# Autodesk Inventor assembly: claws_endeffector_6
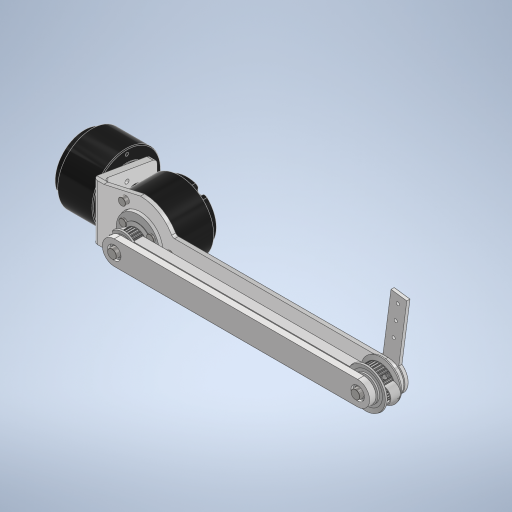
[picture p0: Inventor's stored thumbnail of the model, 512x512]
Saved by Autodesk Inventor 2024 (Build 280153000, 153)
## iProperties
Created: 2025-04-20
Part Number: claws_endeffector_6
Document SubType Name: Assembly
Designer: 1412z
Author: 1412z
## Documents named in this file (17)
- C:\Users\1412z\OneDrive\デスクトップ\rdclab\harvesting_robot\harvesting_endeffector\claws_endeffector\claws_endeffector_6.iam
- C:\Users\1412z\OneDrive\デスクトップ\rdclab\harvesting_robot\harvesting_endeffector\claws_endeffector\motor_holder\motor_holder_6.ipt
- C:\Users\1412z\OneDrive\デスクトップ\rdclab\harvesting_robot\harvesting_endeffector\claws_endeffector\GIM3505-08\GIM3505-8_with-driver.ipt
- C:\Users\1412z\OneDrive\デスクトップ\rdclab\harvesting_robot\harvesting_endeffector\claws_endeffector\misumi\SFL674ZZ_Autodesk_Inventor_2024_20250304\SFL674ZZ.ipt
- C:\Users\1412z\OneDrive\デスクトップ\rdclab\harvesting_robot\harvesting_endeffector\claws_endeffector\misumi\simring\simring_Φ4-Φ5.ipt
- C:\Users\1412z\OneDrive\デスクトップ\rdclab\harvesting_robot\harvesting_endeffector\claws_endeffector\misumi\HTPA22S2M060-A-H4_Autodesk_Inventor_2024_20250419\AIS2024\HTPA22S2M060-A-H4_a-2.ipt
- C:\Users\1412z\OneDrive\デスクトップ\rdclab\harvesting_robot\harvesting_endeffector\claws_endeffector\misumi\M2.5×4\M2.5×4.ipt
- C:\Users\1412z\OneDrive\デスクトップ\rdclab\harvesting_robot\harvesting_endeffector\claws_endeffector\misumi\washer\washer_M4.ipt
- C:\Users\1412z\OneDrive\デスクトップ\rdclab\harvesting_robot\harvesting_endeffector\claws_endeffector\misumi\HTPA32S2M060-A-P4_Autodesk_Inventor_2024_20250419\AIS2024\HTPA32S2M060-A-P4.iam
- C:\Users\1412z\OneDrive\デスクトップ\rdclab\harvesting_robot\harvesting_endeffector\claws_endeffector\motor_holder\motor_holder_top_2.ipt
- C:\Users\1412z\OneDrive\デスクトップ\rdclab\harvesting_robot\harvesting_endeffector\claws_endeffector\cutter_part\cutter_board-2.ipt
- C:\Users\1412z\OneDrive\デスクトップ\rdclab\harvesting_robot\harvesting_endeffector\claws_endeffector\cutter_part\homemade_setcolor-2.ipt
- C:\Users\1412z\OneDrive\デスクトップ\rdclab\harvesting_robot\harvesting_endeffector\claws_endeffector\misumi\shaft\shaft_11.35mm.ipt
- C:\Users\1412z\OneDrive\デスクトップ\rdclab\harvesting_robot\harvesting_endeffector\claws_endeffector\misumi\shaft\shaft_23.3mm.ipt
- C:\Users\1412z\OneDrive\デスクトップ\rdclab\harvesting_robot\harvesting_endeffector\claws_endeffector\misumi\M3×8\M3×8.ipt
- C:\Users\1412z\OneDrive\デスクトップ\rdclab\harvesting_robot\harvesting_endeffector\claws_endeffector\misumi\M3×4\M3×4.ipt
- C:\Users\1412z\OneDrive\デスクトップ\rdclab\harvesting_robot\harvesting_endeffector\claws_endeffector\misumi\HTBN360S2M-60_Inventor\HTBN360S2M-60.ipt
## Components (27 placed, 16 different names)
1. motor_holder_6:1 — 回転:1, 回転:2, 回転:3, 回転:4, 回転:5, 回転:9, 回転:10, 回転:11, 回転:15
2. GIM3505-8_with-driver:1 — 回転:1, 回転:2, 回転:7, 回転:8
3. GIM3505-8_with-driver:2 — 回転:3, 回転:4
4. SFL674ZZ:1 — 回転:5, 回転:6
5. simring_Φ4-Φ5:1 — 回転:6, 回転:23
6. HTPA22S2M060-A-H4_a-2:1 — 回転:7, 回転:8, 回転:12, 回転:13, 回転:14, 回転:18, 回転:30
7. M2.5×4:1 — 回転:10
8. M2.5×4:2 — 回転:12
9. M2.5×4:3 — 回転:14
10. M2.5×4:4 — 回転:11
11. M2.5×4:5 — 回転:13
12. M2.5×4:6 — 回転:9
13. washer_M4:1 — 回転:15, 回転:16
14. HTPA32S2M060-A-P4:1 [sub-assembly] — 回転:16, 回転:17
15. washer_M4:2 — 回転:17, 回転:19
16. washer_M4:3 — 回転:18, 回転:20
17. motor_holder_top_2:1 — 回転:19, 回転:20, 回転:21, 回転:22
18. SFL674ZZ:3 — 回転:21
19. SFL674ZZ:4 — 回転:22, 回転:27
20. cutter_board-2:1 — 回転:23, 回転:24, 回転:25
21. homemade_setcolor-2:1 — 回転:24, 回転:25, 回転:26
22. shaft_11.35mm:1 — 回転:27, 回転:29
23. shaft_23.3mm:1 — 回転:26, 回転:28
24. M3×8:1 — 回転:28
25. M3×4:1 — 回転:29
26. M3×4:2 — 回転:30
27. HTBN360S2M-60:1
## Relationships (30: RevoluteJoint 30)
- 回転:1 [RevoluteJoint]: motor_holder_6:1 ↔ GIM3505-8_with-driver:1
- 回転:2 [RevoluteJoint]: motor_holder_6:1 ↔ GIM3505-8_with-driver:1
- 回転:3 [RevoluteJoint]: motor_holder_6:1 ↔ GIM3505-8_with-driver:2
- 回転:4 [RevoluteJoint]: motor_holder_6:1 ↔ GIM3505-8_with-driver:2
- 回転:5 [RevoluteJoint]: motor_holder_6:1 ↔ SFL674ZZ:1
- 回転:6 [RevoluteJoint]: SFL674ZZ:1 ↔ simring_Φ4-Φ5:1
- 回転:7 [RevoluteJoint]: GIM3505-8_with-driver:1 ↔ HTPA22S2M060-A-H4_a-2:1
- 回転:8 [RevoluteJoint]: GIM3505-8_with-driver:1 ↔ HTPA22S2M060-A-H4_a-2:1
- 回転:9 [RevoluteJoint]: motor_holder_6:1 ↔ M2.5×4:6
- 回転:10 [RevoluteJoint]: motor_holder_6:1 ↔ M2.5×4:1
- 回転:11 [RevoluteJoint]: motor_holder_6:1 ↔ M2.5×4:4
- 回転:12 [RevoluteJoint]: HTPA22S2M060-A-H4_a-2:1 ↔ M2.5×4:2
- 回転:13 [RevoluteJoint]: HTPA22S2M060-A-H4_a-2:1 ↔ M2.5×4:5
- 回転:14 [RevoluteJoint]: HTPA22S2M060-A-H4_a-2:1 ↔ M2.5×4:3
- 回転:15 [RevoluteJoint]: motor_holder_6:1 ↔ washer_M4:1
- 回転:16 [RevoluteJoint]: washer_M4:1 ↔ HTPA32S2M060-A-P4:1
- 回転:17 [RevoluteJoint]: HTPA32S2M060-A-P4:1 ↔ washer_M4:2
- 回転:18 [RevoluteJoint]: HTPA22S2M060-A-H4_a-2:1 ↔ washer_M4:3
- 回転:19 [RevoluteJoint]: washer_M4:2 ↔ motor_holder_top_2:1
- 回転:20 [RevoluteJoint]: washer_M4:3 ↔ motor_holder_top_2:1
- 回転:21 [RevoluteJoint]: motor_holder_top_2:1 ↔ SFL674ZZ:3
- 回転:22 [RevoluteJoint]: motor_holder_top_2:1 ↔ SFL674ZZ:4
- 回転:23 [RevoluteJoint]: simring_Φ4-Φ5:1 ↔ cutter_board-2:1
- 回転:24 [RevoluteJoint]: cutter_board-2:1 ↔ homemade_setcolor-2:1
- 回転:25 [RevoluteJoint]: cutter_board-2:1 ↔ homemade_setcolor-2:1
- 回転:26 [RevoluteJoint]: homemade_setcolor-2:1 ↔ shaft_23.3mm:1
- 回転:27 [RevoluteJoint]: SFL674ZZ:4 ↔ shaft_11.35mm:1
- 回転:28 [RevoluteJoint]: shaft_23.3mm:1 ↔ M3×8:1
- 回転:29 [RevoluteJoint]: shaft_11.35mm:1 ↔ M3×4:1
- 回転:30 [RevoluteJoint]: HTPA22S2M060-A-H4_a-2:1 ↔ M3×4:2
